# Autodesk Inventor assembly: LatSup
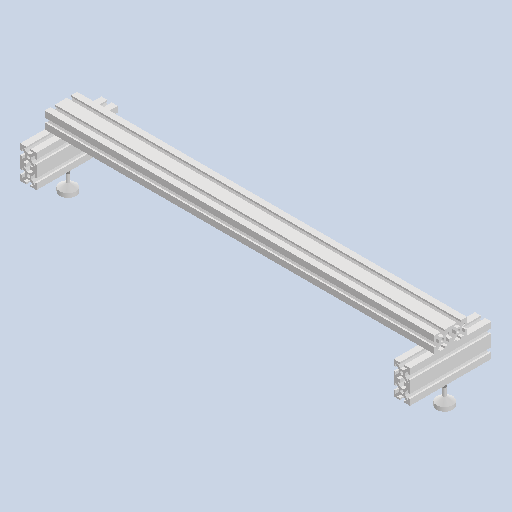
[picture p0: Inventor's stored thumbnail of the model, 512x512]
Saved by Autodesk Inventor 2023 (Build 270158030, 158C)
## iProperties
Created: 2023-02-16
Part Number: LatSup
Document SubType Name: Assembly
Designer: jeremyy
Author: jeremyy
## Documents named in this file (4)
- \\andrew.ad.cmu.edu\users\users1\jeremyy\Documents\Inventor\CMU Bridge\New folder\LatSup.iam
- \\andrew.ad.cmu.edu\users\users1\jeremyy\Documents\Inventor\CMU Bridge\New folder\LatXX24in.ipt
- \\andrew.ad.cmu.edu\users\users1\jeremyy\Documents\Inventor\CMU Bridge\New folder\LongXX5.ipt
- \\andrew.ad.cmu.edu\users\users1\jeremyy\Documents\Inventor\CMU Bridge\New folder\Foot.ipt
## Components (5 placed, 3 different names)
1. LatXX24in:1 — Mate:1, Flush:1, Flush:2, Flush:3, Mate:2, Flush:4
2. LongXX5:1 — Mate:1, Flush:1, Flush:2, Mate:4, Tangent:3, Tangent:4
3. LongXX5:2 — Flush:3, Mate:2, Flush:4, Mate:3, Tangent:1, Tangent:2
4. Foot:1 — Mate:3, Tangent:1, Tangent:2
5. Foot:2 — Mate:4, Tangent:3, Tangent:4
## Relationships (12: Mate 4, Flush 4, Tangent 4)
- Mate:1: LatXX24in:1 ↔ LongXX5:1
- Flush:1: LatXX24in:1 ↔ LongXX5:1
- Flush:2 (-38.1 mm): LatXX24in:1 ↔ LongXX5:1
- Flush:3: LatXX24in:1 ↔ LongXX5:2
- Mate:2: LatXX24in:1 ↔ LongXX5:2
- Flush:4 (-38.1 mm): LatXX24in:1 ↔ LongXX5:2
- Mate:3: LongXX5:2 ↔ Foot:1
- Tangent:1: LongXX5:2 ↔ Foot:1
- Tangent:2 (-63.5 mm): LongXX5:2 ↔ Foot:1
- Mate:4: LongXX5:1 ↔ Foot:2
- Tangent:3: LongXX5:1 ↔ Foot:2
- Tangent:4 (-63.5 mm): LongXX5:1 ↔ Foot:2
